# Autodesk Inventor assembly: F_Foot_v2
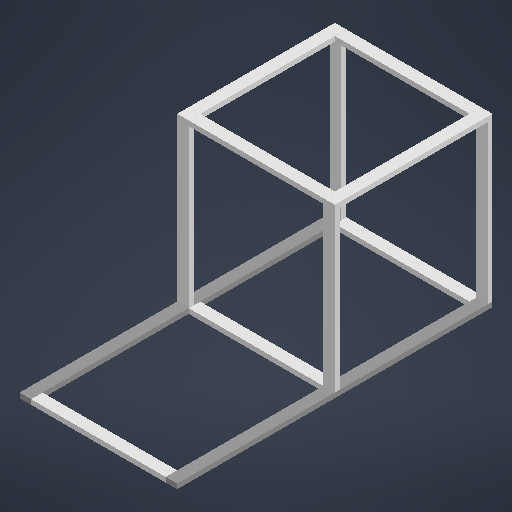
[picture p0: Inventor's stored thumbnail of the model, 512x512]
Saved by Autodesk Inventor 2027.1 (Build 311270010, 270A)
## iProperties
Created: 2026-08-30
Part Number: F_Foot_v2
Document SubType Name: Assembly
Designer: jorda
Author: jorda
## Documents named in this file (4)
- C:\Users\jorda\OneDrive\Documents\GitHub\USC-ASME-TigerBurn-2026\CAD\Legs\Front Foot\F_Foot_v2.iam
- C:\Users\jorda\OneDrive\Documents\GitHub\USC-ASME-TigerBurn-2026\CAD\Legs\Front Foot\2x4x48.ipt
- C:\Users\jorda\OneDrive\Documents\GitHub\USC-ASME-TigerBurn-2026\CAD\Legs\Front Foot\2x4x120.ipt
- C:\Users\jorda\OneDrive\Documents\GitHub\USC-ASME-TigerBurn-2026\CAD\Legs\Front Foot\2x4x41.ipt
## Components (13 placed, 3 different names)
1. 2x4x120:1 — Mate:5, Flush:9, Flush:10, Mate:6, Flush:11, Flush:12
2. 2x4x48:2 — Mate:5, Flush:9, Flush:10, Mate:10, Flush:19, Flush:20
3. 2x4x120:2 — Mate:7, Flush:13, Flush:14, Mate:8, Flush:15, Flush:16, Mate:15, Flush:29
4. 2x4x48:3 — Mate:8, Flush:15, Flush:16, Mate:9, Flush:17, Flush:18
5. 2x4x41:1 — Mate:6, Flush:11, Flush:12
6. 2x4x41:2 — Mate:7, Flush:13, Flush:14
7. 2x4x48:4 — Mate:9, Flush:17, Flush:18, Mate:11, Flush:21, Flush:22, Mate:12, Flush:23, Flush:24, Mate:13, Flush:25, Flush:26
8. 2x4x48:5 — Mate:10, Flush:19, Flush:20, Mate:14, Flush:27, Flush:28
9. 2x4x41:3 — Mate:11, Flush:21, Flush:22
10. 2x4x41:4 — Mate:12, Flush:23, Flush:24
11. 2x4x48:6 — Mate:13, Flush:25, Flush:26, Flush:30
12. 2x4x48:7 — Mate:14, Flush:27, Flush:28
13. 2x4x41:5 — Mate:15, Flush:29, Flush:30
## Relationships (33: Flush 22, Mate 11)
- Mate:5: 2x4x120:1 ↔ 2x4x48:2
- Flush:9: 2x4x120:1 ↔ 2x4x48:2
- Flush:10: 2x4x120:1 ↔ 2x4x48:2
- Mate:6: 2x4x120:1 ↔ 2x4x41:1
- Flush:11: 2x4x120:1 ↔ 2x4x41:1
- Flush:12: 2x4x120:1 ↔ 2x4x41:1
- Mate:7: 2x4x120:2 ↔ 2x4x41:2
- Flush:13: 2x4x120:2 ↔ 2x4x41:2
- Flush:14: 2x4x120:2 ↔ 2x4x41:2
- Mate:8: 2x4x120:2 ↔ 2x4x48:3
- Flush:15: 2x4x120:2 ↔ 2x4x48:3
- Flush:16: 2x4x120:2 ↔ 2x4x48:3
- Mate:9: 2x4x48:3 ↔ 2x4x48:4
- Flush:17: 2x4x48:3 ↔ 2x4x48:4
- Flush:18: 2x4x48:3 ↔ 2x4x48:4
- Mate:10: 2x4x48:2 ↔ 2x4x48:5
- Flush:19: 2x4x48:2 ↔ 2x4x48:5
- Flush:20: 2x4x48:2 ↔ 2x4x48:5
- Mate:11: 2x4x48:4 ↔ 2x4x41:3
- Flush:21: 2x4x48:4 ↔ 2x4x41:3
- Flush:22: 2x4x48:4 ↔ 2x4x41:3
- Mate:12: 2x4x48:4 ↔ 2x4x41:4
- Flush:23: 2x4x48:4 ↔ 2x4x41:4
- Flush:24: 2x4x48:4 ↔ 2x4x41:4
- Mate:13: 2x4x48:4 ↔ 2x4x48:6
- Flush:25: 2x4x48:4 ↔ 2x4x48:6
- Flush:26: 2x4x48:4 ↔ 2x4x48:6
- Mate:14: 2x4x48:5 ↔ 2x4x48:7
- Flush:27: 2x4x48:5 ↔ 2x4x48:7
- Flush:28: 2x4x48:5 ↔ 2x4x48:7
- Mate:15: 2x4x120:2 ↔ 2x4x41:5
- Flush:29: 2x4x120:2 ↔ 2x4x41:5
- Flush:30: 2x4x48:6 ↔ 2x4x41:5
